# Autodesk Inventor assembly: MP1-1001_CAM1
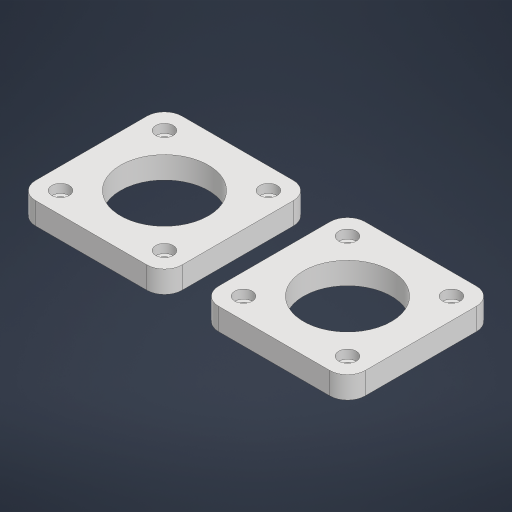
[picture p0: Inventor's stored thumbnail of the model, 512x512]
Saved by Autodesk Inventor 2024.1 (Build 281209000, 209)
## iProperties
Created: 2024-02-20
Part Number: MP1-1001_CAM1
Document SubType Name: Assembly
Designer: fablabadmin
Author: fablabadmin
## Documents named in this file (2)
- C:\Users\fablabadmin\Documents\_Benjamin_S\_3dCAD\HHVerkstad\MountPlate\_CAM\MP1-1001_CAM1_2x.iam
- C:\Users\fablabadmin\Documents\_Benjamin_S\_3dCAD\HHVerkstad\MountPlate\MP1-1001.ipt
## Components (2 placed, 1 different names)
1. MP1-1001:1 — Flush:1, Flush:2, Mate:1
2. MP1-1001:2 — Flush:1, Flush:2, Mate:1
## Relationships (3: Flush 2, Mate 1)
- Flush:1: MP1-1001:1 ↔ MP1-1001:2
- Flush:2: MP1-1001:1 ↔ MP1-1001:2
- Mate:1 (25 mm): MP1-1001:1 ↔ MP1-1001:2
